# Autodesk Inventor assembly: Spool Unit
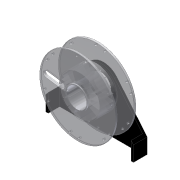
[picture p0: Inventor's stored thumbnail of the model, 180x180]
Saved by Autodesk Inventor 2015 (Build 190159000, 159)
## iProperties
Created: 2018-06-08
Part Number: Spool Unit
Document SubType Name: Assembly
Designer: Ghassan Yusuf
Author: Ghassan Yusuf
## Documents named in this file (3)
- C:\Users\Ghassan Yusuf\Dropbox\MakerBot Transformation\Spool Unit.iam
- C:\Users\Ghassan Yusuf\Dropbox\MakerBot Transformation\filament spool.ipt
- C:\Users\Ghassan Yusuf\Dropbox\MakerBot Transformation\Spool Holder Stand.ipt
## Components (2 placed, 2 different names)
1. filament spool:1 — Insert:1
2. Spool Holder Stand:1 — Insert:1, Flush:1, Flush:2
## Relationships (3: Flush 2, Insert 1)
- Insert:1 (6 mm): filament spool:1 ↔ Spool Holder Stand:1
- Flush:1: Spool Holder Stand:1
- Flush:2: Spool Holder Stand:1
